# Autodesk Inventor assembly: 垃圾桶
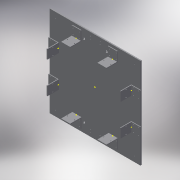
[picture p0: Inventor's stored thumbnail of the model, 180x180]
Saved by Autodesk Inventor 2017 (Build 210142000, 142)
## iProperties
Part Number: 垃圾桶
Material: 常规
Document SubType Name: Assembly
Designer: PANDA
Author: PANDA
## Documents named in this file (3)
- D:\PANDA\Study\VG100\P2\草图\亚克力板\垃圾桶.iam
- D:\PANDA\Study\VG100\P2\草图\亚克力板\上层板.ipt
- D:\PANDA\Study\VG100\P2\草图\亚克力板\连接架.ipt
## Components (9 placed, 2 different names)
1. 上层板:1 — 旋转:1, 旋转:2, 旋转:3, 旋转:4, 旋转:5, 旋转:6, 旋转:7, 旋转:8, 旋转:9, 旋转:10, 旋转:11, 旋转:12, 旋转:13, 旋转:14
2. 连接架:1 — 旋转:3, 旋转:4
3. 连接架:2 — 旋转:5, 旋转:6
4. 连接架:3 — 旋转:11, 旋转:12
5. 连接架:4 — 旋转:13, 旋转:14
6. 连接架:5 — 旋转:1
7. 连接架:6 — 旋转:2
8. 连接架:7 — 旋转:9, 旋转:10
9. 连接架:8 — 旋转:7, 旋转:8
## Relationships (14: RevoluteJoint 14)
- 旋转:1 [RevoluteJoint]: 上层板:1 ↔ 连接架:5
- 旋转:2 [RevoluteJoint]: 上层板:1 ↔ 连接架:6
- 旋转:3 [RevoluteJoint]: 上层板:1 ↔ 连接架:1
- 旋转:4 [RevoluteJoint]: 上层板:1 ↔ 连接架:1
- 旋转:5 [RevoluteJoint]: 上层板:1 ↔ 连接架:2
- 旋转:6 [RevoluteJoint]: 上层板:1 ↔ 连接架:2
- 旋转:7 [RevoluteJoint]: 上层板:1 ↔ 连接架:8
- 旋转:8 [RevoluteJoint]: 上层板:1 ↔ 连接架:8
- 旋转:9 [RevoluteJoint]: 上层板:1 ↔ 连接架:7
- 旋转:10 [RevoluteJoint]: 上层板:1 ↔ 连接架:7
- 旋转:11 [RevoluteJoint]: 上层板:1 ↔ 连接架:3
- 旋转:12 [RevoluteJoint]: 上层板:1 ↔ 连接架:3
- 旋转:13 [RevoluteJoint]: 上层板:1 ↔ 连接架:4
- 旋转:14 [RevoluteJoint]: 上层板:1 ↔ 连接架:4
